# Autodesk Inventor assembly: 66 Tooth Turntable
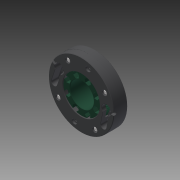
[picture p0: Inventor's stored thumbnail of the model, 180x180]
Saved by Autodesk Inventor 2016 SP2 (Build 200236200, 236)
## iProperties
Created: 2011-04-18
Part Number: 66 Tooth Turntable
Description: STEP AP203
Document SubType Name: Assembly
Designer: Jacob
Sending System: SolidWorks 2010
Preprocessor: SwSTEP 2.0
Title: 276-1810-LARGE.STEP
Revision Number: ANY
## Documents named in this file (6)
- D:\Users\Owner\Desktop\Inventor Files\VEX Parts\Imperial\Motion\66 Tooth Turntable.iam
- D:\Users\Owner\Desktop\Inventor Files\VEX Parts\Imperial\Motion\Components\NUT-832-NYLOCK_ANY.ipt
- D:\Users\Owner\Desktop\Inventor Files\VEX Parts\Imperial\Motion\Components\276-1810-002.ipt
- D:\Users\Owner\Downloads\276-2045-STEP\SCREW-832-0750_ANY.ipt
- D:\Users\Owner\Desktop\Inventor Files\VEX Parts\Imperial\Motion\Components\276-1810-004.ipt
- D:\Users\Owner\Desktop\Inventor Files\VEX Parts\Imperial\Motion\Components\276-1810-003.ipt
## Components (11 placed, 11 different names)
1. NUT-832-NYLOCK_ANY_1 — Mate:5, Mate:6
2. NUT-832-NYLOCK_ANY_2 — Mate:9, Mate:10
3. 276-1810-002_3 — Insert:1
4. SCREW-832-0750_ANY_4 — Insert:4, Mate:10
5. SCREW-832-0750_ANY_5 — Insert:5, Mate:8
6. 276-1810-004_6 — Mate:1, Mate:2, Insert:1, Insert:2, Insert:3, Insert:4, Insert:5
7. NUT-832-NYLOCK_ANY_7 — Mate:3, Mate:4
8. SCREW-832-0750_ANY_8 — Insert:2, Mate:4
9. SCREW-832-0750_ANY_9 — Insert:3, Mate:5
10. 276-1810-003_10 — Mate:1, Mate:2, Mate:3, Mate:6, Mate:7, Mate:9
11. NUT-832-NYLOCK_ANY_11 — Mate:7, Mate:8
## Relationships (15: Mate 10, Insert 5)
- Mate:1: 276-1810-004_6 ↔ 276-1810-003_10
- Mate:2: 276-1810-004_6 ↔ 276-1810-003_10
- Insert:1: 276-1810-002_3 ↔ 276-1810-004_6
- Insert:2: 276-1810-004_6 ↔ SCREW-832-0750_ANY_8
- Insert:3: 276-1810-004_6 ↔ SCREW-832-0750_ANY_9
- Insert:4: SCREW-832-0750_ANY_4 ↔ 276-1810-004_6
- Insert:5: SCREW-832-0750_ANY_5 ↔ 276-1810-004_6
- Mate:3: NUT-832-NYLOCK_ANY_7 ↔ 276-1810-003_10
- Mate:4: NUT-832-NYLOCK_ANY_7 ↔ SCREW-832-0750_ANY_8
- Mate:5: NUT-832-NYLOCK_ANY_1 ↔ SCREW-832-0750_ANY_9
- Mate:6: NUT-832-NYLOCK_ANY_1 ↔ 276-1810-003_10
- Mate:7: 276-1810-003_10 ↔ NUT-832-NYLOCK_ANY_11
- Mate:8: SCREW-832-0750_ANY_5 ↔ NUT-832-NYLOCK_ANY_11
- Mate:9: NUT-832-NYLOCK_ANY_2 ↔ 276-1810-003_10
- Mate:10: NUT-832-NYLOCK_ANY_2 ↔ SCREW-832-0750_ANY_4
